# Autodesk Inventor assembly: Сборка13
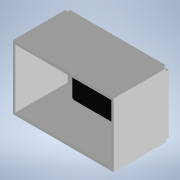
[picture p0: Inventor's stored thumbnail of the model, 180x180]
Saved by Autodesk Inventor 2022 (Build 260153000, 153)
## iProperties
Created: 2023-05-26
Part Number: Сборка13
Document SubType Name: Assembly
Designer: korsh624
Author: korsh624
## Documents named in this file (8)
- C:\git\robot_01\design\Сборка13.iam
- C:\git\robot_01\design\akkum16v.ipt
- C:\git\robot_01\design\akum12v.ipt
- C:\git\robot_01\design\korob\top1.ipt
- C:\git\robot_01\design\goruntu modulu.ipt
- C:\git\robot_01\design\korob\long.ipt
- C:\git\robot_01\design\korob\unlong.ipt
- C:\git\robot_01\design\korob\unlong2.ipt
## Components (8 placed, 7 different names)
1. akkum16v:1 — Заподлицо:4, Совмещение:2, Заподлицо:5, Заподлицо:7, Совмещение:5
2. akum12v:1 — Заподлицо:4, Совмещение:1, Заподлицо:5, Заподлицо:6
3. top1:1 — Совмещение:1, Совмещение:2, Заподлицо:6, Заподлицо:7, Заподлицо:8, Совмещение:3, Заподлицо:9, Заподлицо:10, Совмещение:4, Заподлицо:11, Заподлицо:12
4. goruntu modulu:1 — Заподлицо:8, Совмещение:3, Заподлицо:9
5. long:1 — Заподлицо:10, Заподлицо:14
6. long:2 — Совмещение:4, Заподлицо:11, Заподлицо:12, Совмещение:5, Заподлицо:13
7. unlong:1 — Заподлицо:13
8. unlong2:1 — Заподлицо:14
## Relationships (16: Flush 11, Mate 5)
- Заподлицо:4 [Flush]: akkum16v:1 ↔ akum12v:1
- Совмещение:1 [Mate]: akum12v:1 ↔ top1:1
- Совмещение:2 [Mate]: akkum16v:1 ↔ top1:1
- Заподлицо:5 [Flush]: akkum16v:1 ↔ akum12v:1
- Заподлицо:6 [Flush] (-10 mm): akum12v:1 ↔ top1:1
- Заподлицо:7 [Flush] (15 mm): akkum16v:1 ↔ top1:1
- Заподлицо:8 [Flush]: top1:1 ↔ goruntu modulu:1
- Совмещение:3 [Mate]: top1:1 ↔ goruntu modulu:1
- Заподлицо:9 [Flush] (10 mm): top1:1 ↔ goruntu modulu:1
- Заподлицо:10 [Flush]: top1:1 ↔ long:1
- Совмещение:4 [Mate]: top1:1 ↔ long:2
- Заподлицо:11 [Flush]: top1:1 ↔ long:2
- Заподлицо:12 [Flush]: top1:1 ↔ long:2
- Совмещение:5 [Mate] (10 mm): akkum16v:1 ↔ long:2
- Заподлицо:13 [Flush]: long:2 ↔ unlong:1
- Заподлицо:14 [Flush]: long:1 ↔ unlong2:1
